# Autodesk Inventor assembly: ScissorLift
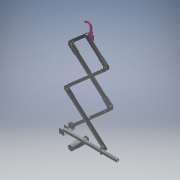
[picture p0: Inventor's stored thumbnail of the model, 180x180]
Saved by Autodesk Inventor 2018.3 (Build 223284000, 284)
## iProperties
Created: 2020-01-12
Part Number: ScissorLift
Document SubType Name: Assembly
Designer: Cooper
Mass: 1637.65 g
Surface Area: 7429.08 cm^2
Volume: 608.716 cm^3
Density: 2.69034 g/cm^3
Author: Cooper
## Documents named in this file (14)
- C:\Users\22perngrac\Documents\GrabCAD\Infinite Recharge 2020\Build season\CLB_026_ScissorLift.iam
- C:\Users\22perngrac\Documents\GrabCAD\Infinite Recharge 2020\Build season\CLB_027_LifterBracket.ipt
- C:\Users\22perngrac\Documents\GrabCAD\Infinite Recharge 2020\Build season\CLB_021_ScissorLiftMotorApproximation.ipt
- C:\Users\22perngrac\Documents\GrabCAD\Infinite Recharge 2020\Build season\CLB_028_ScissorLiftSpacer.ipt
- C:\Users\22perngrac\Documents\GrabCAD\Infinite Recharge 2020\Build season\CLB_029_ScissorLiftBarBottom.ipt
- C:\Users\22perngrac\Documents\GrabCAD\Infinite Recharge 2020\Build season\CLB_034_ScissorLiftBracketOutside.ipt
- C:\Users\22perngrac\Documents\GrabCAD\Infinite Recharge 2020\Build season\CLB_035_ScissorLiftBracketInside.ipt
- C:\Users\22perngrac\Documents\GrabCAD\Infinite Recharge 2020\Build season\CLB_036_ScissorLiftBarTop.ipt
- C:\Users\22perngrac\Documents\GrabCAD\Infinite Recharge 2020\Build season\CLB_037_ScissorLiftBarMiddle.ipt
- C:\Users\22perngrac\Documents\GrabCAD\Infinite Recharge 2020\Build season\CLB_040_ScissorLiftSpacer2.ipt
- C:\Users\22perngrac\Documents\GrabCAD\Infinite Recharge 2020\Build season\CLB_030_ScissorLiftSlider.iam
- C:\Users\22perngrac\Documents\GrabCAD\Infinite Recharge 2020\Build season\CLB_041_ScissorHook.ipt
- C:\Users\22perngrac\Documents\GrabCAD\Infinite Recharge 2020\Build season\CLB_046_ClevisPinScissors.ipt
- C:\Users\22perngrac\Documents\GrabCAD\Infinite Recharge 2020\Build season\CLB_050_ScissorSliderSpacer.ipt
## Components (42 placed, 13 different names)
1. CLB_027_LifterBracket:1 — Mate:30, Flush:97, Mate:129, Symmetry:4
2. CLB_027_LifterBracket:2 — Mate:28, Mate:30, Flush:95, Flush:96, Mate:133, Symmetry:4, Insert:10
3. CLB_027_LifterBracket:3 — Mate:25, Angle:3, Flush:27, Mate:61, Symmetry:5
4. CLB_027_LifterBracket:4 — Mate:25, Angle:3, Mate:28, Flush:28, Mate:96, Symmetry:5
5. CLB_027_LifterBracket:5 — Mate:13, Angle:1, Mate:57, Mate:63, Flush:29, Symmetry:6
6. CLB_027_LifterBracket:6 — Mate:13, Angle:1, Flush:30, Mate:108, Symmetry:6
7. CLB_027_LifterBracket:7 — Mate:18, Mate:57, Flush:100, Mate:123, Symmetry:2, Insert:9
8. CLB_027_LifterBracket:8 — Mate:18, Flush:101, Flush:102, Mate:125, Symmetry:2
9. CLB_027_LifterBracket:9 — Mate:42, Angle:6, Mate:44, Mate:94, Symmetry:7
10. CLB_027_LifterBracket:10 — Mate:41, Angle:7, Angle:11, Flush:32, Mate:86, Symmetry:8
11. CLB_027_LifterBracket:11 — Mate:41, Angle:7, Mate:43, Angle:11, Flush:33, Mate:102, Symmetry:8
12. CLB_027_LifterBracket:12 — Mate:42, Angle:6, Mate:87, Flush:34, Flush:35, Symmetry:7
13. CLB_027_LifterBracket:13 — Mate:36, Angle:5, Mate:44, Flush:93, Mate:132, Symmetry:3, Insert:7
14. CLB_027_LifterBracket:14 — Mate:34, Angle:4, Flush:98, Flush:99, Mate:121, Symmetry:1
15. CLB_027_LifterBracket:15 — Mate:36, Angle:5, Flush:94, Mate:128, Symmetry:3
16. CLB_027_LifterBracket:16 — Mate:34, Angle:4, Mate:43, Mate:118, Symmetry:1, Insert:8
17. CLB_028_ScissorLiftSpacer:1 — Mate:64, Mate:65, Mate:99, Mate:145, Mate:147
18. CLB_029_ScissorLiftBarBottom:1 — Flush:27, Mate:61, Flush:28, Mate:62, Mate:64, Mate:67, Mate:74, Flush:31, Mate:82, Mate:96, Mate:99
19. CLB_029_ScissorLiftBarBottom:2 — Mate:62, Mate:63, Flush:29, Flush:30, Mate:65, Mate:68, Mate:70, Mate:72, Mate:108, Mate:150
20. CLB_030_ScissorLiftSlider:1 [sub-assembly] — Mate:70, Angle:8, Mate:72, Mate:73, Mate:74, Mate:77, Mate:78, Mate:79, Angle:10, Mate:83, Angle:12, Mate:147, Mate:149, Insert:11
21. CLB_021_ScissorLiftMotorApproximation:1 — Mate:77, Mate:78, Flush:31
22. CLB_034_ScissorLiftBracketOutside:1 — Mate:79, Angle:9, Angle:10
23. CLB_035_ScissorLiftBracketInside:1 — Mate:82, Angle:9, Mate:83
24. CLB_036_ScissorLiftBarTop:1 — Flush:32, Mate:86, Flush:33, Mate:102, Mate:142, Mate:144, Mate:146
25. CLB_036_ScissorLiftBarTop:2 — Mate:87, Flush:34, Flush:35, Mate:94, Mate:142, Mate:143
26. CLB_037_ScissorLiftBarMiddle:1 — Flush:98, Flush:99, Flush:100, Flush:101, Flush:102, Mate:109, Mate:115, Mate:117, Flush:103, Flush:104, Mate:120, Flush:105, Flush:106, Mate:122, Flush:107, Flush:108, Mate:124, Flush:109, Flush:110
27. CLB_037_ScissorLiftBarMiddle:2 — Flush:93, Flush:94, Flush:95, Flush:96, Flush:97, Mate:109, Mate:116, Mate:126, Mate:127, Flush:111, Flush:112, Flush:113, Flush:114, Mate:130, Mate:131, Flush:115, Flush:116, Flush:117, Flush:118
28. CLB_041_ScissorHook:1 — Mate:143, Mate:144, Angle:12
29. CLB_028_ScissorLiftSpacer:2 — Mate:115, Mate:116, Mate:145, Mate:146
30. CLB_040_ScissorLiftSpacer2:1 — Mate:117, Flush:103, Flush:104, Mate:118
31. CLB_040_ScissorLiftSpacer2:2 — Mate:120, Flush:105, Flush:106, Mate:121
32. CLB_040_ScissorLiftSpacer2:3 — Mate:122, Flush:107, Flush:108, Mate:123
33. CLB_040_ScissorLiftSpacer2:4 — Mate:124, Flush:109, Flush:110, Mate:125
34. CLB_040_ScissorLiftSpacer2:5 — Mate:126, Flush:111, Flush:113, Mate:129
35. CLB_040_ScissorLiftSpacer2:6 — Mate:127, Flush:112, Flush:114, Mate:128
36. CLB_040_ScissorLiftSpacer2:7 — Mate:130, Flush:116, Flush:118, Mate:132
37. CLB_040_ScissorLiftSpacer2:8 — Mate:131, Flush:115, Flush:117, Mate:133
38. CLB_046_ClevisPinScissors:1 — Insert:7
39. CLB_046_ClevisPinScissors:2 — Insert:9
40. CLB_046_ClevisPinScissors:3 — Insert:8
41. CLB_046_ClevisPinScissors:4 — Insert:10
42. CLB_050_ScissorSliderSpacer:1 — Mate:149, Insert:11, Mate:150
## Relationships (125: Mate 66, Flush 35, Angle 11, Symmetry 8, Insert 5)
- Mate:13: CLB_027_LifterBracket:5 ↔ CLB_027_LifterBracket:6
- Angle:1 (0 deg): CLB_027_LifterBracket:5 ↔ CLB_027_LifterBracket:6
- Mate:18: CLB_027_LifterBracket:7 ↔ CLB_027_LifterBracket:8
- Mate:25: CLB_027_LifterBracket:3 ↔ CLB_027_LifterBracket:4
- Angle:3 (0 deg): CLB_027_LifterBracket:3 ↔ CLB_027_LifterBracket:4
- Mate:28: CLB_027_LifterBracket:2 ↔ CLB_027_LifterBracket:4
- Mate:30: CLB_027_LifterBracket:1 ↔ CLB_027_LifterBracket:2
- Mate:34: CLB_027_LifterBracket:14 ↔ CLB_027_LifterBracket:16
- Angle:4 (0 deg): CLB_027_LifterBracket:14 ↔ CLB_027_LifterBracket:16
- Mate:36: CLB_027_LifterBracket:13 ↔ CLB_027_LifterBracket:15
- Angle:5 (0 deg): CLB_027_LifterBracket:13 ↔ CLB_027_LifterBracket:15
- Mate:41: CLB_027_LifterBracket:10 ↔ CLB_027_LifterBracket:11
- Mate:42: CLB_027_LifterBracket:9 ↔ CLB_027_LifterBracket:12
- Angle:6 (0 deg): CLB_027_LifterBracket:9 ↔ CLB_027_LifterBracket:12
- Angle:7 (0 deg): CLB_027_LifterBracket:10 ↔ CLB_027_LifterBracket:11
- Mate:43: CLB_027_LifterBracket:11 ↔ CLB_027_LifterBracket:16
- Mate:44: CLB_027_LifterBracket:9 ↔ CLB_027_LifterBracket:13
- Mate:57: CLB_027_LifterBracket:5 ↔ CLB_027_LifterBracket:7
- Flush:27 (25.4 mm): CLB_027_LifterBracket:3 ↔ CLB_029_ScissorLiftBarBottom:1
- Mate:61: CLB_027_LifterBracket:3 ↔ CLB_029_ScissorLiftBarBottom:1
- Flush:28: CLB_027_LifterBracket:4 ↔ CLB_029_ScissorLiftBarBottom:1
- Mate:62: CLB_029_ScissorLiftBarBottom:1 ↔ CLB_029_ScissorLiftBarBottom:2
- Mate:63: CLB_027_LifterBracket:5 ↔ CLB_029_ScissorLiftBarBottom:2
- Flush:29 (25.4 mm): CLB_027_LifterBracket:5 ↔ CLB_029_ScissorLiftBarBottom:2
- Flush:30: CLB_027_LifterBracket:6 ↔ CLB_029_ScissorLiftBarBottom:2
- Mate:64: CLB_028_ScissorLiftSpacer:1 ↔ CLB_029_ScissorLiftBarBottom:1
- Mate:65: CLB_028_ScissorLiftSpacer:1 ↔ CLB_029_ScissorLiftBarBottom:2
- Mate:67: CLB_029_ScissorLiftBarBottom:1
- Mate:68: CLB_029_ScissorLiftBarBottom:2
- Mate:70: CLB_029_ScissorLiftBarBottom:2 ↔ CLB_030_ScissorLiftSlider:1
- Angle:8 (0 deg): CLB_030_ScissorLiftSlider:1
- Mate:72 (6.35 mm): CLB_029_ScissorLiftBarBottom:2 ↔ CLB_030_ScissorLiftSlider:1
- Mate:73: CLB_030_ScissorLiftSlider:1
- Mate:74: CLB_029_ScissorLiftBarBottom:1 ↔ CLB_030_ScissorLiftSlider:1
- Mate:77 (-177.8 mm): CLB_030_ScissorLiftSlider:1 ↔ CLB_021_ScissorLiftMotorApproximation:1
- Mate:78: CLB_030_ScissorLiftSlider:1 ↔ CLB_021_ScissorLiftMotorApproximation:1
- Flush:31: CLB_029_ScissorLiftBarBottom:1 ↔ CLB_021_ScissorLiftMotorApproximation:1
- Mate:79: CLB_030_ScissorLiftSlider:1 ↔ CLB_034_ScissorLiftBracketOutside:1
- Mate:82: CLB_029_ScissorLiftBarBottom:1 ↔ CLB_035_ScissorLiftBracketInside:1
- Angle:9 (0 deg): CLB_034_ScissorLiftBracketOutside:1 ↔ CLB_035_ScissorLiftBracketInside:1
- Angle:10 (0 deg): CLB_030_ScissorLiftSlider:1 ↔ CLB_034_ScissorLiftBracketOutside:1
- Mate:83: CLB_030_ScissorLiftSlider:1 ↔ CLB_035_ScissorLiftBracketInside:1
- Angle:11 (0 deg): CLB_027_LifterBracket:10 ↔ CLB_027_LifterBracket:11
- Flush:32 (25.4 mm): CLB_027_LifterBracket:10 ↔ CLB_036_ScissorLiftBarTop:1
- Mate:86: CLB_027_LifterBracket:10 ↔ CLB_036_ScissorLiftBarTop:1
- Flush:33: CLB_027_LifterBracket:11 ↔ CLB_036_ScissorLiftBarTop:1
- Mate:87: CLB_027_LifterBracket:12 ↔ CLB_036_ScissorLiftBarTop:2
- Flush:34 (25.4 mm): CLB_027_LifterBracket:12 ↔ CLB_036_ScissorLiftBarTop:2
- Flush:35: CLB_027_LifterBracket:12 ↔ CLB_036_ScissorLiftBarTop:2
- Flush:93 (25.4 mm): CLB_027_LifterBracket:13 ↔ CLB_037_ScissorLiftBarMiddle:2
- Flush:94: CLB_027_LifterBracket:15 ↔ CLB_037_ScissorLiftBarMiddle:2
- Mate:94: CLB_027_LifterBracket:9 ↔ CLB_036_ScissorLiftBarTop:2
- Flush:95 (25.4 mm): CLB_027_LifterBracket:2 ↔ CLB_037_ScissorLiftBarMiddle:2
- Flush:96: CLB_027_LifterBracket:2 ↔ CLB_037_ScissorLiftBarMiddle:2
- Flush:97: CLB_027_LifterBracket:1 ↔ CLB_037_ScissorLiftBarMiddle:2
- Mate:96: CLB_027_LifterBracket:4 ↔ CLB_029_ScissorLiftBarBottom:1
- Mate:99: CLB_028_ScissorLiftSpacer:1 ↔ CLB_029_ScissorLiftBarBottom:1
- Flush:98 (25.4 mm): CLB_027_LifterBracket:14 ↔ CLB_037_ScissorLiftBarMiddle:1
- Flush:99: CLB_027_LifterBracket:14 ↔ CLB_037_ScissorLiftBarMiddle:1
- Mate:102: CLB_027_LifterBracket:11 ↔ CLB_036_ScissorLiftBarTop:1
- Flush:100: CLB_027_LifterBracket:7 ↔ CLB_037_ScissorLiftBarMiddle:1
- Flush:101: CLB_027_LifterBracket:8 ↔ CLB_037_ScissorLiftBarMiddle:1
- Flush:102 (25.4 mm): CLB_027_LifterBracket:8 ↔ CLB_037_ScissorLiftBarMiddle:1
- Mate:108: CLB_027_LifterBracket:6 ↔ CLB_029_ScissorLiftBarBottom:2
- Mate:109: CLB_037_ScissorLiftBarMiddle:1 ↔ CLB_037_ScissorLiftBarMiddle:2
- Mate:115: CLB_037_ScissorLiftBarMiddle:1 ↔ CLB_028_ScissorLiftSpacer:2
- Mate:116: CLB_037_ScissorLiftBarMiddle:2 ↔ CLB_028_ScissorLiftSpacer:2
- Mate:117: CLB_037_ScissorLiftBarMiddle:1 ↔ CLB_040_ScissorLiftSpacer2:1
- Flush:103: CLB_037_ScissorLiftBarMiddle:1 ↔ CLB_040_ScissorLiftSpacer2:1
- Flush:104: CLB_037_ScissorLiftBarMiddle:1 ↔ CLB_040_ScissorLiftSpacer2:1
- Mate:118: CLB_027_LifterBracket:16 ↔ CLB_040_ScissorLiftSpacer2:1
- Mate:120: CLB_037_ScissorLiftBarMiddle:1 ↔ CLB_040_ScissorLiftSpacer2:2
- Flush:105: CLB_037_ScissorLiftBarMiddle:1 ↔ CLB_040_ScissorLiftSpacer2:2
- Flush:106: CLB_037_ScissorLiftBarMiddle:1 ↔ CLB_040_ScissorLiftSpacer2:2
- Mate:121: CLB_027_LifterBracket:14 ↔ CLB_040_ScissorLiftSpacer2:2
- Mate:122: CLB_037_ScissorLiftBarMiddle:1 ↔ CLB_040_ScissorLiftSpacer2:3
- Flush:107: CLB_037_ScissorLiftBarMiddle:1 ↔ CLB_040_ScissorLiftSpacer2:3
- Flush:108: CLB_037_ScissorLiftBarMiddle:1 ↔ CLB_040_ScissorLiftSpacer2:3
- Mate:123: CLB_027_LifterBracket:7 ↔ CLB_040_ScissorLiftSpacer2:3
- Mate:124: CLB_037_ScissorLiftBarMiddle:1 ↔ CLB_040_ScissorLiftSpacer2:4
- Flush:109: CLB_037_ScissorLiftBarMiddle:1 ↔ CLB_040_ScissorLiftSpacer2:4
- Flush:110: CLB_037_ScissorLiftBarMiddle:1 ↔ CLB_040_ScissorLiftSpacer2:4
- Mate:125: CLB_027_LifterBracket:8 ↔ CLB_040_ScissorLiftSpacer2:4
- Mate:126: CLB_037_ScissorLiftBarMiddle:2 ↔ CLB_040_ScissorLiftSpacer2:5
- Mate:127: CLB_037_ScissorLiftBarMiddle:2 ↔ CLB_040_ScissorLiftSpacer2:6
- Flush:111: CLB_037_ScissorLiftBarMiddle:2 ↔ CLB_040_ScissorLiftSpacer2:5
- Flush:112: CLB_037_ScissorLiftBarMiddle:2 ↔ CLB_040_ScissorLiftSpacer2:6
- Flush:113: CLB_037_ScissorLiftBarMiddle:2 ↔ CLB_040_ScissorLiftSpacer2:5
- Flush:114: CLB_037_ScissorLiftBarMiddle:2 ↔ CLB_040_ScissorLiftSpacer2:6
- Mate:128: CLB_027_LifterBracket:15 ↔ CLB_040_ScissorLiftSpacer2:6
- Mate:129: CLB_027_LifterBracket:1 ↔ CLB_040_ScissorLiftSpacer2:5
- Mate:130: CLB_037_ScissorLiftBarMiddle:2 ↔ CLB_040_ScissorLiftSpacer2:7
- Mate:131: CLB_037_ScissorLiftBarMiddle:2 ↔ CLB_040_ScissorLiftSpacer2:8
- Flush:115: CLB_037_ScissorLiftBarMiddle:2 ↔ CLB_040_ScissorLiftSpacer2:8
- Flush:116: CLB_037_ScissorLiftBarMiddle:2 ↔ CLB_040_ScissorLiftSpacer2:7
- Flush:117: CLB_037_ScissorLiftBarMiddle:2 ↔ CLB_040_ScissorLiftSpacer2:8
- Flush:118: CLB_037_ScissorLiftBarMiddle:2 ↔ CLB_040_ScissorLiftSpacer2:7
- Mate:132: CLB_027_LifterBracket:13 ↔ CLB_040_ScissorLiftSpacer2:7
- Mate:133: CLB_027_LifterBracket:2 ↔ CLB_040_ScissorLiftSpacer2:8
- Symmetry:1: CLB_027_LifterBracket:14 ↔ CLB_027_LifterBracket:16
- Symmetry:2: CLB_027_LifterBracket:7 ↔ CLB_027_LifterBracket:8
- Symmetry:3: CLB_027_LifterBracket:13 ↔ CLB_027_LifterBracket:15
- Symmetry:4: CLB_027_LifterBracket:1 ↔ CLB_027_LifterBracket:2
- Symmetry:5: CLB_027_LifterBracket:3 ↔ CLB_027_LifterBracket:4
- Symmetry:6: CLB_027_LifterBracket:5 ↔ CLB_027_LifterBracket:6
- Symmetry:7: CLB_027_LifterBracket:9 ↔ CLB_027_LifterBracket:12
- Symmetry:8: CLB_027_LifterBracket:10 ↔ CLB_027_LifterBracket:11
- Mate:134
- Mate:135
- Mate:136
- Mate:137
- Mate:142: CLB_036_ScissorLiftBarTop:1 ↔ CLB_036_ScissorLiftBarTop:2
- Mate:143: CLB_036_ScissorLiftBarTop:2 ↔ CLB_041_ScissorHook:1
- Mate:144: CLB_036_ScissorLiftBarTop:1 ↔ CLB_041_ScissorHook:1
- Angle:12 (0 deg): CLB_030_ScissorLiftSlider:1 ↔ CLB_041_ScissorHook:1
- Insert:7: CLB_027_LifterBracket:13 ↔ CLB_046_ClevisPinScissors:1
- Insert:8: CLB_027_LifterBracket:16 ↔ CLB_046_ClevisPinScissors:3
- Insert:9: CLB_027_LifterBracket:7 ↔ CLB_046_ClevisPinScissors:2
- Insert:10: CLB_027_LifterBracket:2 ↔ CLB_046_ClevisPinScissors:4
- Mate:145: CLB_028_ScissorLiftSpacer:1 ↔ CLB_028_ScissorLiftSpacer:2
- Mate:146: CLB_036_ScissorLiftBarTop:1 ↔ CLB_028_ScissorLiftSpacer:2
- Mate:147: CLB_028_ScissorLiftSpacer:1 ↔ CLB_030_ScissorLiftSlider:1
- Mate:149: CLB_030_ScissorLiftSlider:1 ↔ CLB_050_ScissorSliderSpacer:1
- Insert:11: CLB_030_ScissorLiftSlider:1 ↔ CLB_050_ScissorSliderSpacer:1
- Mate:150: CLB_029_ScissorLiftBarBottom:2 ↔ CLB_050_ScissorSliderSpacer:1
